# Autodesk Inventor assembly: DrivePod subassembly
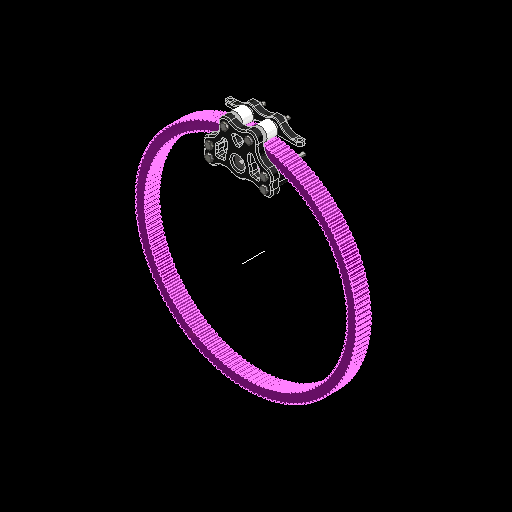
[picture p0: Inventor's stored thumbnail of the model, 512x512]
Saved by Autodesk Inventor 2022 (Build 260153000, 153)
## iProperties
Created: 2022-07-23
Part Number: DrivePod subassembly
Document SubType Name: Assembly
Designer: tandu
Mass: 116.175 g
Surface Area: 485.384 cm^2
Volume: 83.9806 cm^3
Density: 1.38335 g/cm^3
Author: tandu
## Documents named in this file (13)
- C:\Users\tandu\Documents\GrabCAD\3 Pound Leviathan\DrivePod subassembly.iam
- C:\Users\tandu\Documents\GrabCAD\3 Pound Leviathan\CustomTiming Pulley.ipt
- C:\Users\tandu\Documents\GrabCAD\3 Pound Leviathan\DriveTrainPlate.ipt
- C:\Users\tandu\Documents\GrabCAD\3 Pound Leviathan\DriveTrainRoller.ipt
- C:\Users\tandu\Documents\GrabCAD\3 Pound Leviathan\DriveTrainStandoffs.ipt
- C:\Users\tandu\Documents\GrabCAD\3 Pound Leviathan\DriveTrainTopStandoff.ipt
- C:\Users\tandu\Documents\GrabCAD\3 Pound Leviathan\REV-41-1125.ipt
- C:\Users\tandu\Documents\GrabCAD\3 Pound Leviathan\CustomTiming Belt Wheel.ipt
- C:\Users\tandu\Documents\GrabCAD\3 Pound Leviathan\Parameters Part.ipt
- C:\Users\tandu\Documents\GrabCAD\3 Pound Leviathan\Derived Drivepod Plate.ipt
- C:\Users\tandu\Documents\GrabCAD\3 Pound Leviathan\90576A102_Medium-Strength Steel Nylon-Insert Locknut.ipt
- C:\Users\tandu\Documents\GrabCAD\3 Pound Leviathan\Small Drive Bearing 57155K571_Flanged Ball Bearing.ipt
- C:\Users\tandu\Documents\GrabCAD\3 Pound Leviathan\Vex 3 8th nylon roller spacer.ipt
## Components (20 placed, 11 different names)
1. CustomTiming Pulley:1 — Mate:3, Flush:1, Tangent:1, Rotation:1, Mate:5
2. DriveTrainPlate:1
3. DriveTrainRoller:1 — Insert:6
4. DriveTrainStandoffs:1 — Insert:7, Insert:8
5. DriveTrainTopStandoff:1 — Insert:3, Insert:4, Insert:5, Insert:6, Insert:15, Insert:16, Mate:6, Mate:7
6. REV-41-1125:1 — Insert:11
7. CustomTiming Belt Wheel:1 — Mate:1, Mate:2, Flush:1, Tangent:1, Rotation:1, Mate:4
8. Derived Drivepod Plate:1 — Mate:4, Mate:5, Flush:2, Insert:1, Insert:2, Insert:3, Insert:4, Insert:7, Insert:8, Insert:9, Insert:10, Insert:11, Insert:12, Insert:13, Insert:14, Insert:17
9. DriveTrainStandoffs:2 — Insert:1, Insert:2
10. DriveTrainRoller:2 — Insert:5
11. Small Drive Bearing 57155K571_Flanged Ball Bearing:1 — Insert:17
12. Vex 3 8th nylon roller spacer:1 — Mate:7, Mate:9
13. Vex 3 8th nylon roller spacer:2 — Mate:6, Mate:8
14. REV-41-1125:2 — Insert:9
15. REV-41-1125:3 — Insert:10
16. REV-41-1125:4 — Insert:12
17. REV-41-1125:5 — Insert:13
18. REV-41-1125:6 — Insert:14
19. 90576A102_Medium-Strength Steel Nylon-Insert Locknut:1 — Insert:15
20. 90576A102_Medium-Strength Steel Nylon-Insert Locknut:2 — Insert:16
## Relationships (30: Insert 17, Mate 9, Flush 2, Tangent 1, RelateRotation 1)
- Mate:1: CustomTiming Belt Wheel:1
- Mate:2: CustomTiming Belt Wheel:1
- Mate:3: CustomTiming Pulley:1
- Flush:1: CustomTiming Pulley:1 ↔ CustomTiming Belt Wheel:1
- Tangent:1: CustomTiming Pulley:1 ↔ CustomTiming Belt Wheel:1
- Rotation:1 [RelateRotation] (0.1184 ul): CustomTiming Pulley:1 ↔ CustomTiming Belt Wheel:1
- Mate:4 (1.27 mm): CustomTiming Belt Wheel:1 ↔ Derived Drivepod Plate:1
- Mate:5: CustomTiming Pulley:1 ↔ Derived Drivepod Plate:1
- Flush:2: Derived Drivepod Plate:1
- Insert:1: Derived Drivepod Plate:1 ↔ DriveTrainStandoffs:2
- Insert:2: Derived Drivepod Plate:1 ↔ DriveTrainStandoffs:2
- Insert:3: DriveTrainTopStandoff:1 ↔ Derived Drivepod Plate:1
- Insert:4: DriveTrainTopStandoff:1 ↔ Derived Drivepod Plate:1
- Insert:5 (1.27 mm): DriveTrainTopStandoff:1 ↔ DriveTrainRoller:2
- Insert:6 (1.27 mm): DriveTrainRoller:1 ↔ DriveTrainTopStandoff:1
- Insert:7: DriveTrainStandoffs:1 ↔ Derived Drivepod Plate:1
- Insert:8: DriveTrainStandoffs:1 ↔ Derived Drivepod Plate:1
- Insert:9: Derived Drivepod Plate:1 ↔ REV-41-1125:2
- Insert:10: Derived Drivepod Plate:1 ↔ REV-41-1125:3
- Insert:11: REV-41-1125:1 ↔ Derived Drivepod Plate:1
- Insert:12: Derived Drivepod Plate:1 ↔ REV-41-1125:4
- Insert:13: Derived Drivepod Plate:1 ↔ REV-41-1125:5
- Insert:14: Derived Drivepod Plate:1 ↔ REV-41-1125:6
- Insert:15: DriveTrainTopStandoff:1 ↔ 90576A102_Medium-Strength Steel Nylon-Insert Locknut:1
- Insert:16: DriveTrainTopStandoff:1 ↔ 90576A102_Medium-Strength Steel Nylon-Insert Locknut:2
- Insert:17: Derived Drivepod Plate:1 ↔ Small Drive Bearing 57155K571_Flanged Ball Bearing:1
- Mate:6: DriveTrainTopStandoff:1 ↔ Vex 3 8th nylon roller spacer:2
- Mate:7: DriveTrainTopStandoff:1 ↔ Vex 3 8th nylon roller spacer:1
- Mate:8: Vex 3 8th nylon roller spacer:2
- Mate:9: Vex 3 8th nylon roller spacer:1
## Named parameters: WheelThickness = 8.255 mm, WheelDiameter = 381 mm, WheelWidth = 12.7 mm, WheelRatio = 101.6 mm, WallThickness = 6.35 mm, TeethGapLengthMain = 2 mm, TeethDepthMain = 1 mm, TeethStickingOutAdjustment = 0.25 mm, MotorTeeth = 14, WheelTeeth = 152, FixedWheelRatio = 0.118421, TeethInput = 18, TeethInput_1 = 152
